# Autodesk Inventor assembly: Link2
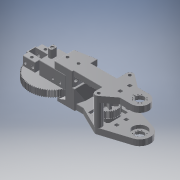
[picture p0: Inventor's stored thumbnail of the model, 180x180]
Saved by Autodesk Inventor 2019 (Build 230136000, 136)
## iProperties
Created: 2020-02-16
Part Number: Link2
Document SubType Name: Assembly
Designer: Alex
Author: Alex
## Documents named in this file (6)
- D:\Alex\Documents\GitHub\RBE3001-URDF-Example\STLs\FinalSTLS\Inventor_Assy\Link2.iam
- D:\Alex\Documents\Personal Projects\BenchPowerSupply\Link2_Frame1.ipt
- D:\Alex\Documents\Personal Projects\BenchPowerSupply\Link2_Frame2.ipt
- D:\Alex\Documents\Personal Projects\BenchPowerSupply\Link2_LoadCellBlock.ipt
- D:\Alex\Documents\Personal Projects\BenchPowerSupply\Link2_DriveGear.ipt
- D:\Alex\Documents\Personal Projects\BenchPowerSupply\Link2_DrivenGear.ipt
## Components (5 placed, 5 different names)
1. Link2_Frame1:1 — Flush:1, Flush:2, Flush:3
2. Link2_Frame2:1 — Flush:4, Flush:5, Flush:6
3. Link2_LoadCellBlock:1 — Flush:7, Flush:8, Flush:9
4. Link2_DriveGear:1 — Flush:13, Flush:14, Flush:15
5. Link2_DrivenGear:1 — Flush:16, Flush:17, Flush:18
## Relationships (15: Flush 15)
- Flush:1: Link2_Frame1:1
- Flush:2: Link2_Frame1:1
- Flush:3: Link2_Frame1:1
- Flush:4: Link2_Frame2:1
- Flush:5: Link2_Frame2:1
- Flush:6: Link2_Frame2:1
- Flush:7: Link2_LoadCellBlock:1
- Flush:8: Link2_LoadCellBlock:1
- Flush:9: Link2_LoadCellBlock:1
- Flush:13: Link2_DriveGear:1
- Flush:14: Link2_DriveGear:1
- Flush:15: Link2_DriveGear:1
- Flush:16: Link2_DrivenGear:1
- Flush:17: Link2_DrivenGear:1
- Flush:18: Link2_DrivenGear:1
